# Autodesk Inventor assembly: Throughput Mockup Assembly
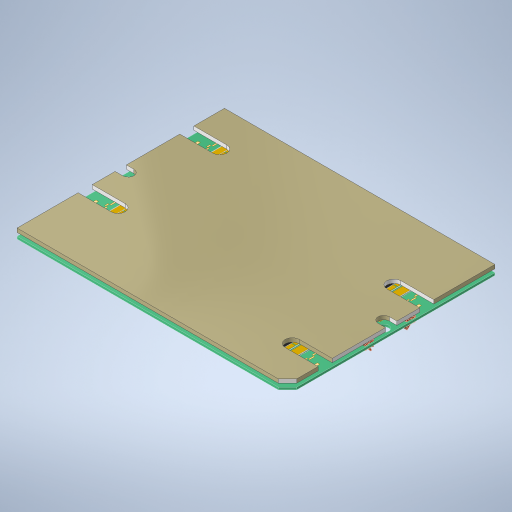
[picture p0: Inventor's stored thumbnail of the model, 512x512]
Saved by Autodesk Inventor 2023 (Build 270158000, 158)
## iProperties
Created: 2022-04-25
Part Number: Throughput Mockup Assembly
Document SubType Name: Assembly
Designer: Caleb
Author: Caleb
## Documents named in this file (7)
- C:\Users\Caleb\Desktop\nebraska-silicon-lab\Hardware\ETL\modules\throughput mockups\Throughput Mockup Assembly.iam
- C:\Users\Caleb\Desktop\nebraska-silicon-lab\Hardware\ETL\modules\throughput mockups\etl_module_pcb_mockup_v3p3etl_module_pcb_mockup_v3p3.iam
- C:\Users\Caleb\Desktop\nebraska-silicon-lab\Hardware\ETL\modules\throughput mockups\BBM Assembly.iam
- C:\Users\Caleb\Desktop\nebraska-silicon-lab\Hardware\ETL\ETL-SH-Design\3D-model\K3D-WP7B-S050VA1-V3_JAE_Proprietary v1_14.iam
- C:\Users\Caleb\Desktop\nebraska-silicon-lab\Hardware\ETL\modules\throughput mockups\Coverplate Film.ipt
- C:\Users\Caleb\Desktop\nebraska-silicon-lab\Hardware\ETL\modules\throughput mockups\Sensor Placement Film.ipt
- C:\Users\Caleb\Desktop\nebraska-silicon-lab\Hardware\ETL\modules\throughput mockups\Baseplate v1.5.ipt
## Components (10 placed, 6 different names)
1. etl_module_pcb_mockup_v3p3:1 [sub-assembly] — Mate:10, Angle:1, Flush:8, Flush:9, Angle:2, Flush:14, Flush:15, Angle:3
2. BBM Assembly:1 [sub-assembly] — Flush:17, Flush:20, Mate:13, Flush:22
3. BBM Assembly:2 [sub-assembly] — Flush:16, Flush:19, Mate:14, Flush:21, Mate:15
4. BBM Assembly:3 [sub-assembly] — Flush:18, Flush:20, Mate:13, Mate:14, Flush:21, Angle:3
5. BBM Assembly:4 [sub-assembly] — Flush:16, Flush:17, Flush:18, Flush:19, Flush:22, Flush:23, Flush:24, Mate:16, Flush:25, Flush:26
6. K3D-WP7B-S050VA1-V3_JAE_Proprietary v1_14:1 [sub-assembly]
7. K3D-WP7B-S050VA1-V3_JAE_Proprietary v1_14:2 [sub-assembly]
8. Coverplate Film:1 — Angle:2, Mate:12, Mate:16, Flush:25, Flush:26
9. Sensor Placement Film:1 — Mate:10, Angle:1, Flush:8, Flush:9, Mate:15, Flush:23, Flush:24
10. Baseplate v1.5:1 — Mate:12, Flush:14, Flush:15
## Relationships (24: Flush 15, Mate 6, Angle 3)
- Mate:10: etl_module_pcb_mockup_v3p3:1 ↔ Sensor Placement Film:1
- Angle:1 (0 deg): etl_module_pcb_mockup_v3p3:1 ↔ Sensor Placement Film:1
- Flush:8 (0.75 mm): etl_module_pcb_mockup_v3p3:1 ↔ Sensor Placement Film:1
- Flush:9 (5.45 mm): etl_module_pcb_mockup_v3p3:1 ↔ Sensor Placement Film:1
- Angle:2 (0 deg): etl_module_pcb_mockup_v3p3:1 ↔ Coverplate Film:1
- Mate:12: Coverplate Film:1 ↔ Baseplate v1.5:1
- Flush:14: etl_module_pcb_mockup_v3p3:1 ↔ Baseplate v1.5:1
- Flush:15: etl_module_pcb_mockup_v3p3:1 ↔ Baseplate v1.5:1
- Flush:16: BBM Assembly:2 ↔ BBM Assembly:4
- Flush:17: BBM Assembly:1 ↔ BBM Assembly:4
- Flush:18: BBM Assembly:3 ↔ BBM Assembly:4
- Flush:19: BBM Assembly:2 ↔ BBM Assembly:4
- Flush:20: BBM Assembly:1 ↔ BBM Assembly:3
- Mate:13 (0.2 mm): BBM Assembly:1 ↔ BBM Assembly:3
- Mate:14 (0.2 mm): BBM Assembly:2 ↔ BBM Assembly:3
- Flush:21: BBM Assembly:2 ↔ BBM Assembly:3
- Flush:22: BBM Assembly:1 ↔ BBM Assembly:4
- Mate:15: BBM Assembly:2 ↔ Sensor Placement Film:1
- Angle:3 (0 deg): etl_module_pcb_mockup_v3p3:1 ↔ BBM Assembly:3
- Flush:23: BBM Assembly:4 ↔ Sensor Placement Film:1
- Flush:24: BBM Assembly:4 ↔ Sensor Placement Film:1
- Mate:16: BBM Assembly:4 ↔ Coverplate Film:1
- Flush:25 (0.5 mm): BBM Assembly:4 ↔ Coverplate Film:1
- Flush:26 (0.9 mm): BBM Assembly:4 ↔ Coverplate Film:1
